# Autodesk Inventor assembly: DB2_Bridge_Assembly
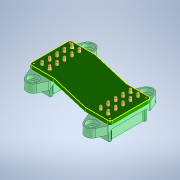
[picture p0: Inventor's stored thumbnail of the model, 180x180]
Saved by Autodesk Inventor 2021 (Build 250183000, 183)
## iProperties
Created: 2020-04-05
Part Number: DB2_Bridge_Assembly
Document SubType Name: Assembly
Designer: lgnds
Author: lgnds
## Documents named in this file (3)
- C:\Users\lgnds\Documents\GitHub\WaveRunner-CCU\CCU_Assembly\hw\CAD\DB2_Bridge_Assembly.iam
- C:\Users\lgnds\Documents\GitHub\WaveRunner-CCU\CCU_Assembly\hw\CAD\PCB\DB2_Bridge.ipt
- C:\Users\lgnds\Documents\GitHub\WaveRunner-CCU\CCU_Assembly\hw\CAD\Other\m300-fv3104500_asm\m300-fv3104500_asm.iam
## Components (3 placed, 2 different names)
1. DB2_Bridge:1 — Mate:1, Mate:2, Mate:3, Mate:4, Mate:5, Mate:6
2. m300-fv3104500_asm:1 [sub-assembly] — Mate:1, Mate:2, Mate:3
3. m300-fv3104500_asm:2 [sub-assembly] — Mate:4, Mate:5, Mate:6
## Relationships (6: Mate 6)
- Mate:1: DB2_Bridge:1 ↔ m300-fv3104500_asm:1
- Mate:2: DB2_Bridge:1 ↔ m300-fv3104500_asm:1
- Mate:3: DB2_Bridge:1 ↔ m300-fv3104500_asm:1
- Mate:4: DB2_Bridge:1 ↔ m300-fv3104500_asm:2
- Mate:5: DB2_Bridge:1 ↔ m300-fv3104500_asm:2
- Mate:6: DB2_Bridge:1 ↔ m300-fv3104500_asm:2
